# Autodesk Inventor assembly: back_platform_assembly
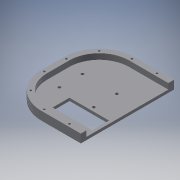
[picture p0: Inventor's stored thumbnail of the model, 180x180]
Saved by Autodesk Inventor 2016 (Build 200138000, 138)
## iProperties
Created: 2015-09-09
Part Number: back_platform_assembly
Document SubType Name: Assembly
Designer: oscar
Author: oscar
## Documents named in this file (3)
- C:\Users\oscar\Desktop\technical_drawings\youbot\back_platform\v1.0\inventor_parts\back_platform_assembly.iam
- C:\Users\oscar\Desktop\technical_drawings\youbot\back_platform\v1.0\inventor_parts\back_platform.ipt
- C:\Users\oscar\Desktop\technical_drawings\youbot\back_platform\v1.0\inventor_parts\side_walls.ipt
## Components (5 placed, 2 different names)
1. back_platform:1 — Mate:1, Mate:3, Flush:3, Mate:4, Flush:4, Flush:5, Mate:5, Flush:8, Flush:9
2. side_walls:1 — Mate:2, Flush:1, Flush:2
3. side_walls:2 — Mate:1, Mate:2, Flush:1, Flush:2, Flush:4, Flush:5
4. side_walls:3 — Mate:6, Flush:6, Flush:7
5. side_walls:4 — Mate:5, Mate:6, Flush:6, Flush:7, Flush:8, Flush:9
## Relationships (15: Flush 9, Mate 6)
- Mate:1: back_platform:1 ↔ side_walls:2
- Mate:2: side_walls:1 ↔ side_walls:2
- Flush:1: side_walls:1 ↔ side_walls:2
- Flush:2: side_walls:1 ↔ side_walls:2
- Mate:3: back_platform:1
- Flush:3: back_platform:1
- Mate:4: back_platform:1
- Flush:4: back_platform:1 ↔ side_walls:2
- Flush:5: back_platform:1 ↔ side_walls:2
- Mate:5: back_platform:1 ↔ side_walls:4
- Mate:6: side_walls:3 ↔ side_walls:4
- Flush:6: side_walls:3 ↔ side_walls:4
- Flush:7: side_walls:3 ↔ side_walls:4
- Flush:8: back_platform:1 ↔ side_walls:4
- Flush:9: back_platform:1 ↔ side_walls:4
